# Autodesk Inventor assembly: finish_assembly_1
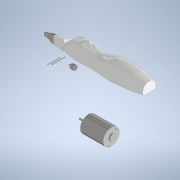
[picture p0: Inventor's stored thumbnail of the model, 180x180]
Saved by Autodesk Inventor 2020 (Build 240168000, 168)
## iProperties
Created: 2020-02-11
Part Number: finish_assembly_1
Document SubType Name: Assembly
Designer: metal
Author: metal
## Documents named in this file (10)
- C:\Polyimide_isolation_cleaner\finish_assembly_1.iam
- C:\Polyimide_isolation_cleaner\korob_3.ipt
- C:\Polyimide_isolation_cleaner\pielers2.ipt
- C:\Polyimide_isolation_cleaner\pielers.ipt
- C:\Polyimide_isolation_cleaner\plastic_case_back_4.ipt
- C:\Polyimide_isolation_cleaner\курок.ipt
- C:\Polyimide_isolation_cleaner\excentrick_2.ipt
- C:\Polyimide_isolation_cleaner\направляющая.ipt
- C:\Polyimide_isolation_cleaner\R370-25120.ipt
- C:\Polyimide_isolation_cleaner\blade.ipt
## Components (12 placed, 9 different names)
1. korob_3:1 — Rigid:1, Slider:1
2. pielers2:1 — Rotational:1, Rigid:9
3. pielers:1 — Rigid:1, Rotational:1, Rigid:10
4. plastic_case_back_4:1 — Rigid:11, Slider:1
5. курок:1 — Rotational:3
6. excentrick_2:1
7. направляющая:3 — Rigid:11, Rotational:3
8. направляющая:4
9. R370-25120:1
10. blade:1 — Rigid:10
11. blade:2 — Rigid:9
12. направляющая:5
## Relationships (7: WeldJoint 4, RevoluteJoint 2, TranslationJoint 1)
- Rigid:1 [WeldJoint]: korob_3:1 ↔ pielers:1
- Rotational:1 [RevoluteJoint] (-0.4 mm): pielers2:1 ↔ pielers:1
- Rigid:9 [WeldJoint]: pielers2:1 ↔ blade:2
- Rigid:10 [WeldJoint]: pielers:1 ↔ blade:1
- Rigid:11 [WeldJoint]: plastic_case_back_4:1 ↔ направляющая:3
- Rotational:3 [RevoluteJoint]: курок:1 ↔ направляющая:3
- Slider:1 [TranslationJoint]: korob_3:1 ↔ plastic_case_back_4:1
